# Autodesk Inventor assembly: ExteriorBumperCar
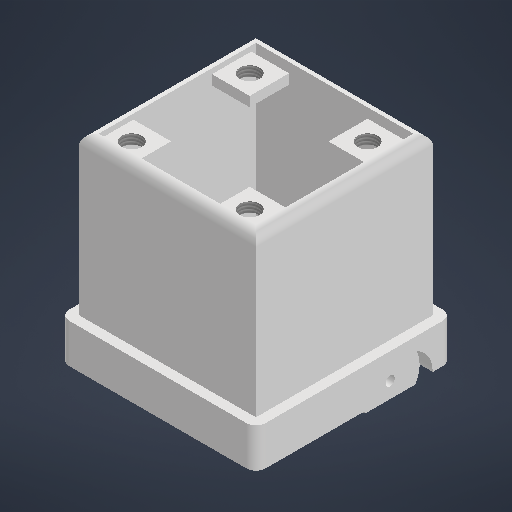
[picture p0: Inventor's stored thumbnail of the model, 512x512]
Saved by Autodesk Inventor 2026.1 (Build 301233000, 233)
## iProperties
Created: 2026-06-28
Part Number: ExteriorBumperCar
Document SubType Name: Assembly
Designer: Kasi Pusuluri
Author: Kasi Pusuluri
## Documents named in this file (6)
- C:\Users\Kasi Pusuluri\Documents\Outpost 2026\CAD\BumperCar\ExteriorBumperCar.iam
- C:\Users\Kasi Pusuluri\Documents\Outpost 2026\BumperCarV2\BumperBody.ipt
- C:\Users\Kasi Pusuluri\Documents\Outpost 2026\BumperCarV2\Connector1.ipt
- C:\Users\Kasi Pusuluri\Documents\Outpost 2026\BumperCarV2\MotorProtector.ipt
- C:\Users\Kasi Pusuluri\Documents\Outpost 2026\BumperCarV2\Base.ipt
- C:\Users\Kasi Pusuluri\Documents\Outpost 2026\BumperCarV2\WheelConnector.ipt
## Components (10 placed, 5 different names)
1. BumperBody:1 — Rigid:1, Rigid:2, Mate:1, Mate:2
2. Connector1:1
3. Connector1:2
4. Connector1:3
5. Connector1:4
6. MotorProtector:1 — Rigid:1
7. MotorProtector:2 — Rigid:2
8. Base:1 — Mate:1, Mate:2
9. WheelConnector:1
10. WheelConnector:2
## Relationships (4: WeldJoint 2, Mate 2)
- Rigid:1 [WeldJoint]: BumperBody:1 ↔ MotorProtector:1
- Rigid:2 [WeldJoint]: BumperBody:1 ↔ MotorProtector:2
- Mate:1: BumperBody:1 ↔ Base:1
- Mate:2: BumperBody:1 ↔ Base:1
